# Autodesk Inventor assembly: P1699_EG
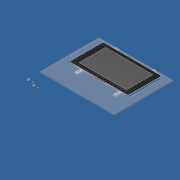
[picture p0: Inventor's stored thumbnail of the model, 180x180]
Saved by Autodesk Inventor 2015 SP2 (Build 190223200, 223)
## iProperties
Created: 2017-06-14
Part Number: P1699_EG
Project: Nom Projet
Description: Ens. Nom Ensemble
Document SubType Name: Assembly
Designer: Francis-Lucien-Hugue
Author: Francis-Lucien-Hugue
## Documents named in this file (7)
- C:\Users\Francis-Lucien-Hugue\Desktop\TimbreuseLocal\hardware\box\P1699_EG.iam
- C:\Users\Francis-Lucien-Hugue\Desktop\TimbreuseLocal\hardware\box\Box.ipt
- C:\Users\Francis-Lucien-Hugue\Desktop\TimbreuseLocal\hardware\box\P1699_002_FaceAvant.ipt
- C:\Users\Francis-Lucien-Hugue\Desktop\TimbreuseLocal\hardware\box\Imported Components\Raspberry_Pi_Touch_Screen_Assembly_-_Pins_Out\Raspberry_Pi_Touch_Screen_Assembly_-_Pins_Out.iam
- C:\Users\Francis-Lucien-Hugue\Desktop\TimbreuseLocal\hardware\box\P1699_003_Support.ipt
- C:\Users\Francis-Lucien-Hugue\Documents\Inventor\Content Center Files\R2015\fr-FR\DIN 912\DIN 912 - M3 x 0.5 x 8 x 6.75.ipt
- C:\Users\Francis-Lucien-Hugue\Documents\Inventor\Content Center Files\R2015\fr-FR\DIN 912\DIN 912 - M3 x 0.5 x 12 x 10.75.ipt
## Components (13 placed, 5 different names)
1. Box:1 — Placage:1, Placage:2, Placage:3
2. Pièce1:1 — Placage:1, Placage:2, Placage:3, Placage:4, Placage:5, Placage:6, Placage:7, Logement:5, Logement:6
3. Raspberry_Pi_Touch_Screen_Assembly_-_Pins_Out:1 [sub-assembly] — Placage:8, Placage:9, Placage:10, Placage:11, Placage:12, Placage:13
4. Pièce1:2 — Placage:6, Placage:7, Placage:8, Placage:9, Placage:12, Logement:1, Logement:2
5. Pièce1:3 — Placage:4, Placage:5, Placage:10, Placage:11, Placage:13, Logement:3, Logement:4
6. DIN 912 - Remplacé par DIN EN ISO 4762 M3 x 8:1 — Logement:2
7. DIN 912 - Remplacé par DIN EN ISO 4762 M3 x 8:2 — Logement:4
8. DIN 912 - Remplacé par DIN EN ISO 4762 M3 x 8:3 — Logement:1
9. DIN 912 - Remplacé par DIN EN ISO 4762 M3 x 8:4 — Logement:3
10. DIN 912 - Remplacé par DIN EN ISO 4762 M3 x 12:1
11. DIN 912 - Remplacé par DIN EN ISO 4762 M3 x 12:2
12. DIN 912 - Remplacé par DIN EN ISO 4762 M3 x 12:3 — Logement:6
13. DIN 912 - Remplacé par DIN EN ISO 4762 M3 x 12:4 — Logement:5
## Relationships (19: Mate 13, Insert 6)
- Placage:1 [Mate]: Box:1 ↔ Pièce1:1
- Placage:2 [Mate]: Box:1 ↔ Pièce1:1
- Placage:3 [Mate]: Box:1 ↔ Pièce1:1
- Placage:4 [Mate]: Pièce1:1 ↔ Pièce1:3
- Placage:5 [Mate]: Pièce1:1 ↔ Pièce1:3
- Placage:6 [Mate]: Pièce1:1 ↔ Pièce1:2
- Placage:7 [Mate]: Pièce1:1 ↔ Pièce1:2
- Placage:8 [Mate]: Raspberry_Pi_Touch_Screen_Assembly_-_Pins_Out:1 ↔ Pièce1:2
- Placage:9 [Mate]: Raspberry_Pi_Touch_Screen_Assembly_-_Pins_Out:1 ↔ Pièce1:2
- Placage:10 [Mate]: Raspberry_Pi_Touch_Screen_Assembly_-_Pins_Out:1 ↔ Pièce1:3
- Placage:11 [Mate]: Raspberry_Pi_Touch_Screen_Assembly_-_Pins_Out:1 ↔ Pièce1:3
- Placage:12 [Mate]: Raspberry_Pi_Touch_Screen_Assembly_-_Pins_Out:1 ↔ Pièce1:2
- Placage:13 [Mate]: Raspberry_Pi_Touch_Screen_Assembly_-_Pins_Out:1 ↔ Pièce1:3
- Logement:1 [Insert]: Pièce1:2 ↔ DIN 912 - Remplacé par DIN EN ISO 4762 M3 x 8:3
- Logement:2 [Insert]: Pièce1:2 ↔ DIN 912 - Remplacé par DIN EN ISO 4762 M3 x 8:1
- Logement:3 [Insert]: Pièce1:3 ↔ DIN 912 - Remplacé par DIN EN ISO 4762 M3 x 8:4
- Logement:4 [Insert]: Pièce1:3 ↔ DIN 912 - Remplacé par DIN EN ISO 4762 M3 x 8:2
- Logement:5 [Insert]: Pièce1:1 ↔ DIN 912 - Remplacé par DIN EN ISO 4762 M3 x 12:4
- Logement:6 [Insert]: Pièce1:1 ↔ DIN 912 - Remplacé par DIN EN ISO 4762 M3 x 12:3
